# Autodesk Inventor assembly: GFRP_T3_03
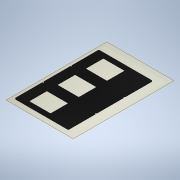
[picture p0: Inventor's stored thumbnail of the model, 180x180]
Saved by Autodesk Inventor 2020 (Build 240168000, 168)
## iProperties
Created: 2021-08-27
Part Number: GFRP_T3_03
Document SubType Name: Assembly
Designer: Masato
Author: Masato
## Documents named in this file (3)
- D:\GitHub\inventor\SUSTAINA-OP\Cam\GFRP_T3_03.iam
- D:\GitHub\inventor\SUSTAINA-OP\Cam\DisposableBoard.ipt
- D:\GitHub\inventor\SUSTAINA-OP\LowerBody\Foot\Sole_frame.ipt
## Components (4 placed, 2 different names)
1. DisposableBoard:1 — メイト:2, メイト:1, フラッシュ:1, フラッシュ:2, メイト:4, メイト:5, メイト:6
2. Sole_frame:1 — メイト:4, メイト:5, メイト:6
3. Sole_frame:2
4. Sole_frame:3
## Component patterns: (3 elements, first: Sole_frame:1)
## Relationships (7: Mate 5, Flush 2)
- メイト:2 [Mate]: DisposableBoard:1
- メイト:1 [Mate]: DisposableBoard:1
- フラッシュ:1 [Flush]: DisposableBoard:1
- フラッシュ:2 [Flush]: DisposableBoard:1
- メイト:4 [Mate]: DisposableBoard:1 ↔ Sole_frame:1
- メイト:5 [Mate] (2 mm): DisposableBoard:1 ↔ Sole_frame:1
- メイト:6 [Mate] (2 mm): DisposableBoard:1 ↔ Sole_frame:1
